# Autodesk Inventor assembly: Head
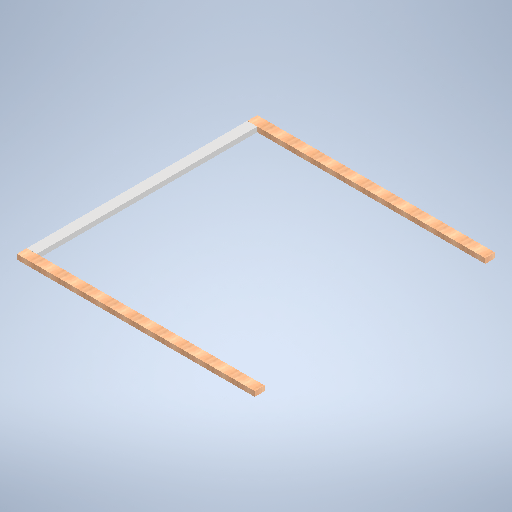
[picture p0: Inventor's stored thumbnail of the model, 512x512]
Saved by Autodesk Inventor 2025 (Build 290162000, 162)
## iProperties
Created: 2024-09-18
Part Number: Head
Document SubType Name: Assembly
Designer: localadmin
Author: localadmin
## Documents named in this file (3)
- C:\Users\localadmin\Documents\USCTigerBurn24\Head.iam
- C:\Users\localadmin\Documents\USCTigerBurn24\Standard Timber\2x4x96.ipt
- C:\Users\localadmin\Documents\USCTigerBurn24\Standard Timber\7'5''x2x4.ipt
## Components (3 placed, 2 different names)
1. 2x4x96:1 — Flush:1, Flush:2, Mate:1
2. 2x4x96:2 — Flush:1, Flush:2, Mate:1, Flush:3, Flush:4
3. 7'5''x2x4:1 — Flush:3, Flush:4
## Relationships (5: Flush 4, Mate 1)
- Flush:1: 2x4x96:1 ↔ 2x4x96:2
- Flush:2: 2x4x96:1 ↔ 2x4x96:2
- Mate:1 (2260.6 mm): 2x4x96:1 ↔ 2x4x96:2
- Flush:3: 2x4x96:2 ↔ 7'5''x2x4:1
- Flush:4: 2x4x96:2 ↔ 7'5''x2x4:1
